# Autodesk Inventor assembly: Ensamblaje1
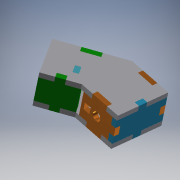
[picture p0: Inventor's stored thumbnail of the model, 180x180]
Saved by Autodesk Inventor 2018 (Build 220112000, 112)
## iProperties
Created: 2020-03-13
Part Number: Ensamblaje1
Material: Genérico
Document SubType Name: Assembly
Designer: joser
Author: joser
## Documents named in this file (8)
- C:\Users\joser\OneDrive\Escritorio\Parte alvaro\Ensamblaje1.iam
- C:\Users\joser\OneDrive\Escritorio\Parte alvaro\Lateral.ipt
- C:\Users\joser\OneDrive\Escritorio\Parte alvaro\Barilla.ipt
- C:\Users\joser\OneDrive\Escritorio\Parte alvaro\back.ipt
- C:\Users\joser\OneDrive\Escritorio\Parte alvaro\Top.ipt
- C:\Users\joser\OneDrive\Escritorio\Parte alvaro\Top1.ipt
- C:\Users\joser\OneDrive\Escritorio\Parte alvaro\abajo.ipt
- C:\Users\joser\OneDrive\Escritorio\Parte alvaro\abajo1.ipt
## Components (8 placed, 7 different names)
1. Lateral:1 — Coincidencia:1, Coincidencia:3, Coincidencia:4
2. Barilla:1 — Coincidencia:1, Coincidencia:3, Coincidencia:4, Coincidencia:5, Coincidencia:6, Coincidencia:7, Coincidencia:8, Coincidencia:9, Coincidencia:10
3. Lateral:2 — Coincidencia:5, Coincidencia:6, Coincidencia:7, Coincidencia:14, Coincidencia:15, Coincidencia:16, Coincidencia:17, Coincidencia:18, Coincidencia:19, Coincidencia:20, Coincidencia:21, Coincidencia:22
4. back:1 — Coincidencia:8, Coincidencia:9, Coincidencia:10, Coincidencia:11, Coincidencia:12, Coincidencia:13
5. Top:1 — Coincidencia:11, Coincidencia:12, Coincidencia:13
6. Top1:1 — Coincidencia:14, Coincidencia:15, Coincidencia:16
7. abajo:1 — Coincidencia:17, Coincidencia:18, Coincidencia:19
8. abajo1:1 — Coincidencia:20, Coincidencia:21, Coincidencia:22
## Relationships (21: Mate 21)
- Coincidencia:1 [Mate]: Lateral:1 ↔ Barilla:1
- Coincidencia:3 [Mate]: Lateral:1 ↔ Barilla:1
- Coincidencia:4 [Mate]: Lateral:1 ↔ Barilla:1
- Coincidencia:5 [Mate]: Barilla:1 ↔ Lateral:2
- Coincidencia:6 [Mate]: Barilla:1 ↔ Lateral:2
- Coincidencia:7 [Mate]: Barilla:1 ↔ Lateral:2
- Coincidencia:8 [Mate]: Barilla:1 ↔ back:1
- Coincidencia:9 [Mate]: Barilla:1 ↔ back:1
- Coincidencia:10 [Mate]: Barilla:1 ↔ back:1
- Coincidencia:11 [Mate]: back:1 ↔ Top:1
- Coincidencia:12 [Mate]: back:1 ↔ Top:1
- Coincidencia:13 [Mate]: back:1 ↔ Top:1
- Coincidencia:14 [Mate]: Lateral:2 ↔ Top1:1
- Coincidencia:15 [Mate]: Lateral:2 ↔ Top1:1
- Coincidencia:16 [Mate]: Lateral:2 ↔ Top1:1
- Coincidencia:17 [Mate]: Lateral:2 ↔ abajo:1
- Coincidencia:18 [Mate]: Lateral:2 ↔ abajo:1
- Coincidencia:19 [Mate]: Lateral:2 ↔ abajo:1
- Coincidencia:20 [Mate]: Lateral:2 ↔ abajo1:1
- Coincidencia:21 [Mate]: Lateral:2 ↔ abajo1:1
- Coincidencia:22 [Mate]: Lateral:2 ↔ abajo1:1
